# Autodesk Inventor assembly: 吊架-短(R)(#01.05) - 焊接組合_MIR
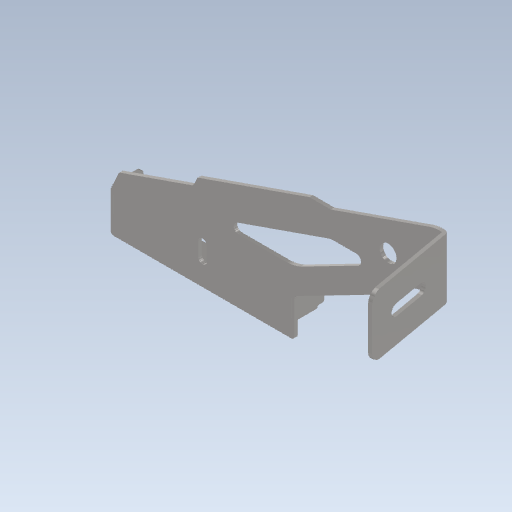
[picture p0: Inventor's stored thumbnail of the model, 512x512]
Saved by Autodesk Inventor 2020 (Build 240168000, 168)
## iProperties
Created: 2015-11-28
Part Number: 吊架-短(R)(#01.05) - 焊接組合_MIR
Document SubType Name: Assembly
Designer: 德國牧羊犬
Author: 設計製圖
## Documents named in this file (3)
- D:\資料庫\設計-3D Project\【May club 】\得利卡-車頂燈架\模型、圖面\短-車頂燈架-組合(#01.05)\吊架-短(R)(#01.05) - 焊接組合_MIR.iam
- D:\資料庫\設計-3D Project\【May club 】\得利卡-車頂燈架\模型、圖面\短-車頂燈架-組合(#01.05)\吊架-短(R)#01.05)- 焊接件-1_MIR.ipt
- D:\資料庫\設計-3D Project\【May club 】\得利卡-車頂燈架\模型、圖面\短-車頂燈架-組合(#01.05)\吊架-短(#01.05) - 焊接件-2_MIR.ipt
## Components (2 placed, 2 different names)
1. 吊架-短(R)#01.05)- 焊接件-1_MIR:1 — 貼合:3, 貼合:2, 貼合:1
2. 吊架-短(#01.05) - 焊接件-2_MIR:1 — 貼合:3, 貼合:2, 貼合:1
## Relationships (3: Mate 2, Flush 1)
- 貼合:3 [Mate]: 吊架-短(R)#01.05)- 焊接件-1_MIR:1 ↔ 吊架-短(#01.05) - 焊接件-2_MIR:1
- 貼合:2 [Flush]: 吊架-短(R)#01.05)- 焊接件-1_MIR:1 ↔ 吊架-短(#01.05) - 焊接件-2_MIR:1
- 貼合:1 [Mate]: 吊架-短(R)#01.05)- 焊接件-1_MIR:1 ↔ 吊架-短(#01.05) - 焊接件-2_MIR:1
